# Autodesk Inventor assembly: Ensamblaje
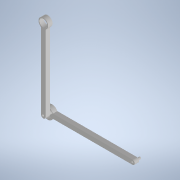
[picture p0: Inventor's stored thumbnail of the model, 180x180]
Saved by Autodesk Inventor 2021 (Build 250183000, 183)
## iProperties
Created: 2022-10-24
Part Number: Ensamblaje
Document SubType Name: Assembly
Designer: ivanm
Author: ivanm
## Documents named in this file (3)
- C:\Users\ivanm\OneDrive\Servomecanismos\Proyectos\Proyecto academico\Servomecanismo2R\INVENTOR\Ensamblaje.iam
- C:\Users\ivanm\OneDrive\Servomecanismos\Proyectos\Proyecto academico\Servomecanismo2R\INVENTOR\eslabon1.ipt
- C:\Users\ivanm\OneDrive\Servomecanismos\Proyectos\Proyecto academico\Servomecanismo2R\INVENTOR\eslabon2.ipt
## Components (2 placed, 2 different names)
1. eslabon1:1 — De rotación:1
2. eslabon2:1 — De rotación:1
## Relationships (1: RevoluteJoint 1)
- De rotación:1 [RevoluteJoint]: eslabon1:1 ↔ eslabon2:1
